# Autodesk Inventor assembly: Mecanismo
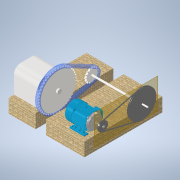
[picture p0: Inventor's stored thumbnail of the model, 180x180]
Saved by Autodesk Inventor 2020 (Build 240168000, 168)
## iProperties
Created: 2021-01-07
Part Number: Mecanismo
Document SubType Name: Assembly
Designer: DanielAlvaradoPelaez
Author: DanielAlvaradoPelaez
## Documents named in this file (10)
- C:\Users\User\Desktop\diseño y simulacion\Archivo Bryan\proyecto2\Mecanismo.iam
- C:\Users\User\Desktop\diseño y simulacion\Archivo Bryan\proyecto2\Pieza1.ipt
- C:\Users\User\Desktop\diseño y simulacion\Archivo Bryan\proyecto2\Pieza2.ipt
- C:\Users\User\Desktop\diseño y simulacion\Archivo Bryan\proyecto2\Pieza4.ipt
- C:\Users\User\Desktop\diseño y simulacion\Archivo Bryan\proyecto2\Pieza3.ipt
- C:\Users\User\Desktop\diseño y simulacion\Archivo Bryan\proyecto2\Pieza5.ipt
- C:\Users\User\Desktop\diseño y simulacion\Archivo Bryan\proyecto2\Mecanismo\Design Accelerator\Transmisión de correa trapezoidal1.iam
- C:\Users\User\Desktop\diseño y simulacion\Archivo Bryan\proyecto2\eje.iam
- C:\Users\User\Desktop\diseño y simulacion\Archivo Bryan\proyecto2\Maquina de bolas.iam
- C:\Users\User\Desktop\diseño y simulacion\Archivo Bryan\proyecto2\Mecanismo\Design Accelerator\Transmisión por cadena1.iam
## Components (9 placed, 9 different names)
1. Pieza1:1 — Coincidencia:3, Coincidencia:4, Coincidencia:5, Coincidencia:7, Coincidencia:8, Nivelación:1, Nivelación:2
2. Pieza2:1 — Coincidencia:6, Coincidencia:7
3. Pieza4:1 — Coincidencia:1, Coincidencia:2, Coincidencia:6, Ángulo:1
4. Pieza3:1 — Coincidencia:1, Coincidencia:2, Coincidencia:3, Coincidencia:4, Coincidencia:5
5. Pieza5:1 — Coincidencia:8, Nivelación:1, Nivelación:2, Ángulo:1, Nivelación:3, Coincidencia:9, Ángulo:2
6. Transmisión de correa trapezoidal:1 [sub-assembly] — Insertar:1, Nivelación:5, Nivelación:6
7. eje:1 [sub-assembly] — Insertar:1
8. Maquina de bolas:1 [sub-assembly] — Nivelación:3, Nivelación:4
9. Transmisión por cadena:1 [sub-assembly]
## Relationships (18: Mate 9, Flush 6, Angle 2, Insert 1)
- Coincidencia:1 [Mate]: Pieza4:1 ↔ Pieza3:1
- Coincidencia:2 [Mate]: Pieza4:1 ↔ Pieza3:1
- Coincidencia:3 [Mate]: Pieza1:1 ↔ Pieza3:1
- Coincidencia:4 [Mate]: Pieza1:1 ↔ Pieza3:1
- Coincidencia:5 [Mate]: Pieza1:1 ↔ Pieza3:1
- Coincidencia:6 [Mate]: Pieza2:1 ↔ Pieza4:1
- Coincidencia:7 [Mate]: Pieza1:1 ↔ Pieza2:1
- Coincidencia:8 [Mate]: Pieza1:1 ↔ Pieza5:1
- Nivelación:1 [Flush] (60 mm): Pieza1:1 ↔ Pieza5:1
- Nivelación:2 [Flush] (60 mm): Pieza1:1 ↔ Pieza5:1
- Ángulo:1 [Angle] (0 deg): Pieza4:1 ↔ Pieza5:1
- Insertar:1: Transmisión de correa trapezoidal:1 ↔ eje:1
- Nivelación:3 [Flush]: Pieza5:1 ↔ Maquina de bolas:1
- Coincidencia:9 [Mate]: Pieza5:1
- Ángulo:2 [Angle] (90 deg): Pieza5:1
- Nivelación:4 [Flush]: Maquina de bolas:1
- Nivelación:5 [Flush]: Transmisión de correa trapezoidal:1
- Nivelación:6 [Flush]: Transmisión de correa trapezoidal:1
